# Autodesk Inventor assembly: REV-41-1600
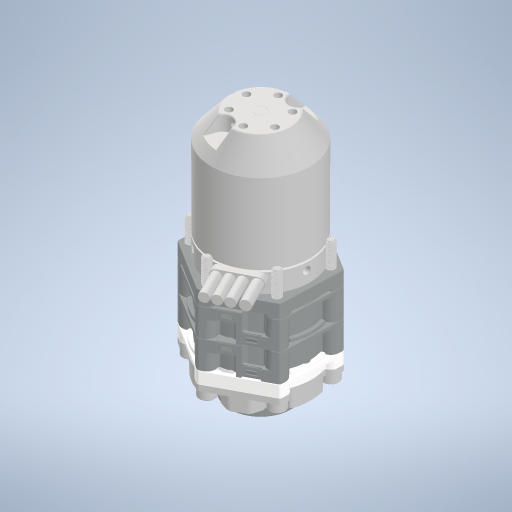
[picture p0: Inventor's stored thumbnail of the model, 512x512]
Saved by Autodesk Inventor 2023.3 (Build 273359000, 359)
## iProperties
Created: 2019-08-05
Part Number: REV-41-1600
Description: STEP AP214
Document SubType Name: Assembly
Designer: jackc
Title: REV-41-1600.STEP
Revision Number: ANY
Sending System: SolidWorks 2018
Preprocessor: SwSTEP 2.0
## Documents named in this file (8)
- C:\Users\jackc\OneDrive\CAD\Parametric Turret\Gears and Pulleys\UltraPlanetary\REV-41-1600.iam
- C:\Users\jackc\OneDrive\CAD\Parametric Turret\Gears and Pulleys\UltraPlanetary\REV-41-1607.ipt
- C:\Users\jackc\OneDrive\CAD\Parametric Turret\Gears and Pulleys\UltraPlanetary\M3x8 Button Head_91239A113.ipt
- C:\Users\jackc\OneDrive\CAD\Parametric Turret\Gears and Pulleys\UltraPlanetary\REV-41-1603.iam
- C:\Users\jackc\OneDrive\CAD\Parametric Turret\Gears and Pulleys\UltraPlanetary\REV-41-1601.iam
- C:\Users\jackc\OneDrive\CAD\Parametric Turret\Gears and Pulleys\UltraPlanetary\REV-41-1604.iam
- C:\Users\jackc\OneDrive\CAD\Parametric Turret\Gears and Pulleys\UltraPlanetary\M3X40_91290A136.ipt
- C:\Users\jackc\OneDrive\CAD\Parametric Turret\Motors\REV-21-1651.ipt
## Components (13 placed, 13 different names)
1. REV-41-1607_2 — Mate:1, Mate:2, Mate:18, Mate:19, Mate:20, Mate:21, Mate:22
2. M3x8 Button Head_91239A113_3 — Mate:2, Mate:16
3. REV-41-1603_5 [sub-assembly] — Mate:11, Mate:12, Mate:15, Mate:22
4. REV-41-1601_7 [sub-assembly] — Mate:10, Mate:11, Mate:13, Mate:14
5. M3x8 Button Head_91239A113_8 — Mate:1, Mate:17
6. REV-41-1604_9 [sub-assembly] — Mate:3, Mate:4, Mate:5, Mate:6, Mate:7, Mate:8, Mate:9, Mate:10
7. M3X40_91290A136_10 — Flush:4, Mate:7, Mate:14, Mate:15
8. M3X40_91290A136_11 — Flush:1, Mate:3, Flush:5, Mate:5, Mate:20
9. M3X40_91290A136_12 — Flush:2, Flush:3, Mate:9
10. M3X40_91290A136_13 — Flush:1, Mate:6
11. M3X40_91290A136_14 — Flush:2, Flush:5, Mate:4, Mate:12, Mate:13
12. M3X40_91290A136_15 — Flush:3, Flush:4, Mate:8, Mate:21
13. REV-21-1651:1 — Mate:16, Mate:17, Mate:18, Mate:19
## Relationships (27: Mate 22, Flush 5)
- Mate:1: REV-41-1607_2 ↔ M3x8 Button Head_91239A113_8
- Mate:2: REV-41-1607_2 ↔ M3x8 Button Head_91239A113_3
- Flush:1: M3X40_91290A136_11 ↔ M3X40_91290A136_13
- Flush:2: M3X40_91290A136_12 ↔ M3X40_91290A136_14
- Flush:3: M3X40_91290A136_12 ↔ M3X40_91290A136_15
- Flush:4: M3X40_91290A136_10 ↔ M3X40_91290A136_15
- Mate:3: REV-41-1604_9 ↔ M3X40_91290A136_11
- Flush:5: M3X40_91290A136_11 ↔ M3X40_91290A136_14
- Mate:4: REV-41-1604_9 ↔ M3X40_91290A136_14
- Mate:5: REV-41-1604_9 ↔ M3X40_91290A136_11
- Mate:6: REV-41-1604_9 ↔ M3X40_91290A136_13
- Mate:7: REV-41-1604_9 ↔ M3X40_91290A136_10
- Mate:8: REV-41-1604_9 ↔ M3X40_91290A136_15
- Mate:9: REV-41-1604_9 ↔ M3X40_91290A136_12
- Mate:10: REV-41-1601_7 ↔ REV-41-1604_9
- Mate:11: REV-41-1603_5 ↔ REV-41-1601_7
- Mate:12: REV-41-1603_5 ↔ M3X40_91290A136_14
- Mate:13: REV-41-1601_7 ↔ M3X40_91290A136_14
- Mate:14: REV-41-1601_7 ↔ M3X40_91290A136_10
- Mate:15: REV-41-1603_5 ↔ M3X40_91290A136_10
- Mate:16: M3x8 Button Head_91239A113_3 ↔ REV-21-1651:1
- Mate:17: M3x8 Button Head_91239A113_8 ↔ REV-21-1651:1
- Mate:18: REV-41-1607_2 ↔ REV-21-1651:1
- Mate:19: REV-41-1607_2 ↔ REV-21-1651:1
- Mate:20: REV-41-1607_2 ↔ M3X40_91290A136_11
- Mate:21: REV-41-1607_2 ↔ M3X40_91290A136_15
- Mate:22: REV-41-1607_2 ↔ REV-41-1603_5
